# Autodesk Inventor assembly: SCARA
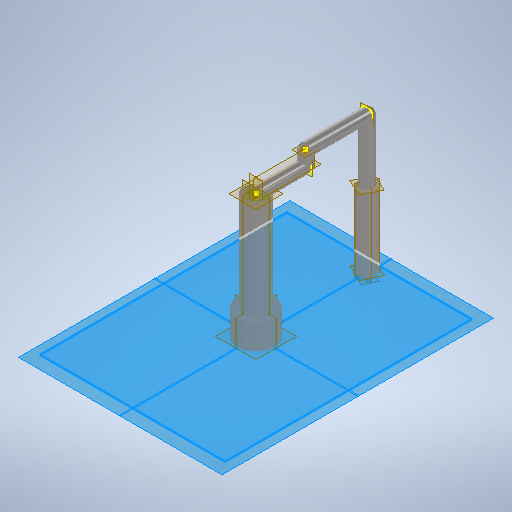
[picture p0: Inventor's stored thumbnail of the model, 512x512]
Saved by Autodesk Inventor 2025.2 (Build 292293000, 293)
## iProperties
Created: 2025-03-23
Part Number: SCARA
Document SubType Name: Assembly
Designer: MSIGAMING
Author: MSIGAMING
## Documents named in this file (8)
- D:\One Drive Manuel\OneDrive\21 Master APE\II Semester\Robotik\3d_robotik\SCARA.iam
- D:\One Drive Manuel\OneDrive\21 Master APE\II Semester\Robotik\3d_robotik\Z0.ipt
- D:\One Drive Manuel\OneDrive\21 Master APE\II Semester\Robotik\3d_robotik\Z1.ipt
- D:\One Drive Manuel\OneDrive\21 Master APE\II Semester\Robotik\3d_robotik\Z2.ipt
- D:\One Drive Manuel\OneDrive\21 Master APE\II Semester\Robotik\3d_robotik\Z3.ipt
- D:\One Drive Manuel\OneDrive\21 Master APE\II Semester\Robotik\3d_robotik\Z4.ipt
- D:\One Drive Manuel\OneDrive\21 Master APE\II Semester\Robotik\3d_robotik\Z5.ipt
- D:\One Drive Manuel\OneDrive\21 Master APE\II Semester\Robotik\3d_robotik\ground.ipt
## Components (7 placed, 7 different names)
1. Z0:1 — Rotational:1, Mate:1, Flush:1, Mate:2
2. Z1:1 — Rotational:1, Flush:2, Mate:3, Mate:4
3. Z2:1 — Flush:2, Mate:3, Mate:4, Mate:5, Mate:6, Mate:7
4. Z3:1 — Mate:5, Mate:6, Mate:7, Rotational:2, Mate:9
5. Z4:1 — Rotational:2, Rotational:3, Mate:8
6. Z5:1 — Rotational:3, Mate:8, Angle:1
7. ground:1 — Mate:10, Flush:3, Mate:11
## Relationships (18: Mate 11, RevoluteJoint 3, Flush 3, Angle 1)
- Rotational:1 [RevoluteJoint]: Z0:1 ↔ Z1:1
- Mate:1: Z0:1
- Flush:1: Z0:1
- Mate:2: Z0:1
- Flush:2: Z1:1 ↔ Z2:1
- Mate:3: Z1:1 ↔ Z2:1
- Mate:4: Z1:1 ↔ Z2:1
- Mate:5: Z2:1 ↔ Z3:1
- Mate:6: Z2:1 ↔ Z3:1
- Mate:7: Z2:1 ↔ Z3:1
- Rotational:2 [RevoluteJoint]: Z3:1 ↔ Z4:1
- Rotational:3 [RevoluteJoint]: Z4:1 ↔ Z5:1
- Mate:8: Z4:1 ↔ Z5:1
- Mate:9: Z3:1
- Mate:10: ground:1
- Flush:3: ground:1
- Mate:11: ground:1
- Angle:1 (0 deg): Z5:1
